# Autodesk Inventor assembly: Assembly1
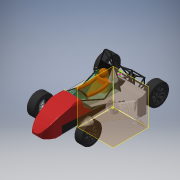
[picture p0: Inventor's stored thumbnail of the model, 180x180]
Saved by Autodesk Inventor 2018.1 (Build 221171000, 171)
## iProperties
Created: 2017-11-07
Part Number: Assembly1
Material: 一般
Document SubType Name: Assembly
Designer: formula
Author: formula
## Documents named in this file (3)
- Z:\各班フォルダ\2018\ボディ\カウル\AeroCAD2018\CAD\Inventor\Aero Parts\Side Pontoon\type2\Assembly1.iam
- Z:\各班フォルダ\2018\ボディ\カウル\AeroCAD2018\CAD\Inventor\Assembly(KS-14.ver)\KS-14_SLow\KS-14_SLow.iam
- Z:\各班フォルダ\2018\ボディ\カウル\AeroCAD2018\CAD\Inventor\Aero Parts\Side Pontoon\type2\parts\ishispe.ipt
## Components (2 placed, 2 different names)
1. KS-14_SLow:1 [sub-assembly] — メイト:1, メイト:2, メイト:3, フラッシュ:2
2. ishispe:1 — メイト:5, フラッシュ:1, フラッシュ:2
## Relationships (6: Mate 4, Flush 2)
- メイト:1 [Mate]: KS-14_SLow:1
- メイト:2 [Mate]: KS-14_SLow:1
- メイト:3 [Mate]: KS-14_SLow:1
- メイト:5 [Mate]: ishispe:1
- フラッシュ:1 [Flush]: ishispe:1
- フラッシュ:2 [Flush]: KS-14_SLow:1 ↔ ishispe:1
